# Autodesk Inventor assembly: PreliminaryDesignR1
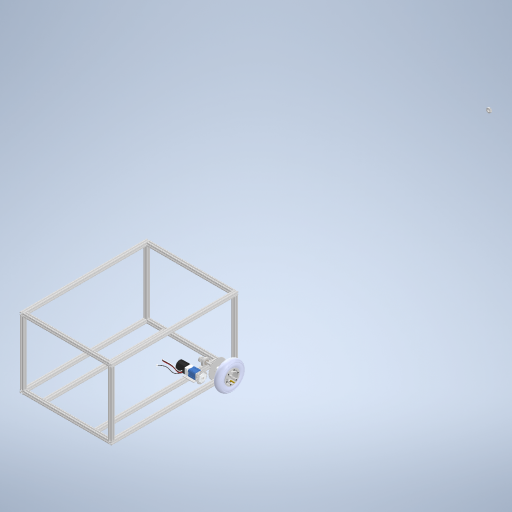
[picture p0: Inventor's stored thumbnail of the model, 512x512]
Saved by Autodesk Inventor 2023 (Build 270158000, 158)
## iProperties
Created: 2022-09-11
Part Number: PreliminaryDesignR1
Document SubType Name: Assembly
Designer: PC
Author: PC
## Documents named in this file (16)
- C:\Users\PC\Documents\PersonalCAD\ARCIGVC\IGVC-Robot\PreliminaryDesignR1.iam
- C:\Users\PC\Documents\PersonalCAD\ARCIGVC\IGVC-Robot\2ft80-20.ipt
- C:\Users\PC\Documents\PersonalCAD\ARCIGVC\IGVC-Robot\3ft80-20.ipt
- C:\Users\PC\Documents\PersonalCAD\ARCIGVC\IGVC-Robot\18in80-20.ipt
- C:\Users\PC\Documents\PersonalCAD\ARCIGVC\IGVC-Robot\34in80-20.ipt
- C:\Users\PC\Documents\PersonalCAD\ARCIGVC\IGVC-Robot\8inPneumatic.ipt
- C:\Users\PC\Documents\PersonalCAD\ARCIGVC\IGVC-Robot\2 Stage HD - CIM Sport.ipt
- C:\Users\PC\Documents\PersonalCAD\ARCIGVC\IGVC-Robot\am-4258 NEO Brushless Motor.ipt
- C:\Users\PC\Documents\PersonalCAD\ARCIGVC\IGVC-Robot\MotorMount.ipt
- C:\Users\PC\Documents\PersonalCAD\ARCIGVC\IGVC-Robot\24tSprocket35Series.ipt
- C:\Users\PC\Documents\PersonalCAD\ARCIGVC\IGVC-Robot\42tSprocket35Series.ipt
- C:\Users\PC\Documents\PersonalCAD\ARCIGVC\IGVC-Robot\Hex Hub .5In.ipt
- C:\Users\PC\Documents\PersonalCAD\ARCIGVC\IGVC-Robot\Bearing Housing.ipt
- C:\Users\PC\Documents\PersonalCAD\ARCIGVC\IGVC-Robot\HalfInHex Bearing.ipt
- C:\Users\PC\Documents\PersonalCAD\ARCIGVC\IGVC-Robot\9in-0.5inHexAxel.ipt
- C:\Users\PC\Documents\PersonalCAD\ARCIGVC\IGVC-Robot\am-1526 500Hex HD Collar Clamp.ipt
## Components (31 placed, 15 different names)
1. 2ft80-20:1 — Mate:1, Flush:1, Flush:2, Flush:4, Mate:4, Flush:7
2. 3ft80-20:1 — Mate:1, Flush:1, Flush:2, Mate:3, Flush:5, Flush:6, Mate:8, Flush:14, Flush:15, Mate:9, Flush:16, Flush:17
3. 2ft80-20:2 — Mate:3, Flush:5, Flush:6, Mate:13, Flush:24, Mate:14, Flush:25
4. 3ft80-20:2 — Flush:4, Mate:4, Flush:7, Mate:10, Flush:18, Flush:19, Mate:11, Flush:20, Flush:21, Mate:29, Flush:29, Mate:43, Mate:44, Mate:45
5. 2ft80-20:3
6. 3ft80-20:3
7. 2ft80-20:4
8. 3ft80-20:4 — Mate:12, Flush:22, Flush:23
9. 18in80-20:1 — Mate:8, Flush:14, Flush:15
10. 18in80-20:2 — Mate:9, Flush:16, Flush:17
11. 18in80-20:3 — Mate:11, Flush:20, Flush:21, Mate:12, Flush:22, Flush:23
12. 18in80-20:4 — Mate:10, Flush:18, Flush:19
13. 34in80-20:1 — Mate:13, Flush:24, Mate:21, Flush:26, Mate:30, Flush:28
14. 34in80-20:2 — Mate:14, Flush:25
15. 8inPneumatic:1 — Mate:41, Mate:43, Mate:45, Flush:31, Mate:48
16. 2 Stage HD - CIM Sport:1 — Mate:15, Mate:16, Mate:17, Mate:18, Mate:19, Mate:20, Mate:25, Flush:27, Mate:44
17. am-4258 NEO Brushless Motor:1 — Mate:15, Mate:16, Mate:17
18. MotorMount:1 — Mate:18, Mate:19, Mate:20, Mate:21, Flush:26, Mate:52
19. 24tSprocket35Series:1 — Mate:22, Mate:23, Mate:24, Flush:30
20. 42tSprocket35Series:1 — Mate:26, Mate:27, Mate:28, Flush:30
21. Hex Hub .5In:1 — Mate:26, Mate:27, Mate:28, Mate:42, Mate:46, Mate:47
22. Hex Hub .5In:2 — Mate:22, Mate:23, Mate:24, Mate:25, Flush:27
23. Bearing Housing:1 — Mate:29, Flush:29, Mate:31, Mate:32, Mate:33, Mate:35, Mate:36, Mate:41, Mate:42
24. Bearing Housing:2 — Mate:30, Flush:28, Mate:31, Mate:37, Mate:38, Mate:39, Mate:40, Mate:52
25. HalfInHex Bearing:1 — Mate:32, Mate:33
26. HalfInHex Bearing:2 — Mate:35, Mate:36
27. HalfInHex Bearing:3 — Mate:37, Mate:40
28. HalfInHex Bearing:4 — Mate:38, Mate:39
29. 9in-0.5inHexAxel:1 — Mate:46, Mate:47, Flush:31, Mate:48, Mate:50, Mate:51
30. am-1526 500Hex HD Collar Clamp:1
31. am-1526 500Hex HD Collar Clamp:2 — Mate:50, Mate:51
## Relationships (79: Mate 49, Flush 30)
- Mate:1: 2ft80-20:1 ↔ 3ft80-20:1
- Flush:1: 2ft80-20:1 ↔ 3ft80-20:1
- Flush:2: 2ft80-20:1 ↔ 3ft80-20:1
- Flush:4: 2ft80-20:1 ↔ 3ft80-20:2
- Mate:3: 3ft80-20:1 ↔ 2ft80-20:2
- Flush:5: 3ft80-20:1 ↔ 2ft80-20:2
- Flush:6: 3ft80-20:1 ↔ 2ft80-20:2
- Mate:4: 2ft80-20:1 ↔ 3ft80-20:2
- Flush:7: 2ft80-20:1 ↔ 3ft80-20:2
- [Mate]: 2ft80-20:3 ↔ 3ft80-20:3
- [Flush]: 2ft80-20:3 ↔ 3ft80-20:3
- [Flush]: 2ft80-20:3 ↔ 3ft80-20:3
- [Flush]: 2ft80-20:3 ↔ 3ft80-20:4
- [Mate]: 3ft80-20:3 ↔ 2ft80-20:4
- [Flush]: 3ft80-20:3 ↔ 2ft80-20:4
- [Flush]: 3ft80-20:3 ↔ 2ft80-20:4
- [Mate]: 2ft80-20:3 ↔ 3ft80-20:4
- [Flush]: 2ft80-20:3 ↔ 3ft80-20:4
- Mate:8: 3ft80-20:1 ↔ 18in80-20:1
- Flush:14: 3ft80-20:1 ↔ 18in80-20:1
- Flush:15: 3ft80-20:1 ↔ 18in80-20:1
- Mate:9: 3ft80-20:1 ↔ 18in80-20:2
- Flush:16: 3ft80-20:1 ↔ 18in80-20:2
- Flush:17: 3ft80-20:1 ↔ 18in80-20:2
- Mate:10: 3ft80-20:2 ↔ 18in80-20:4
- Flush:18: 3ft80-20:2 ↔ 18in80-20:4
- Flush:19: 3ft80-20:2 ↔ 18in80-20:4
- Mate:11: 3ft80-20:2 ↔ 18in80-20:3
- Flush:20: 3ft80-20:2 ↔ 18in80-20:3
- Flush:21: 3ft80-20:2 ↔ 18in80-20:3
- Mate:12: 3ft80-20:4 ↔ 18in80-20:3
- Flush:22: 3ft80-20:4 ↔ 18in80-20:3
- Flush:23: 3ft80-20:4 ↔ 18in80-20:3
- Mate:13: 2ft80-20:2 ↔ 34in80-20:1
- Flush:24: 2ft80-20:2 ↔ 34in80-20:1
- Mate:14: 2ft80-20:2 ↔ 34in80-20:2
- Flush:25: 2ft80-20:2 ↔ 34in80-20:2
- Mate:15: 2 Stage HD - CIM Sport:1 ↔ am-4258 NEO Brushless Motor:1
- Mate:16: 2 Stage HD - CIM Sport:1 ↔ am-4258 NEO Brushless Motor:1
- Mate:17: 2 Stage HD - CIM Sport:1 ↔ am-4258 NEO Brushless Motor:1
- Mate:18: 2 Stage HD - CIM Sport:1 ↔ MotorMount:1
- Mate:19: 2 Stage HD - CIM Sport:1 ↔ MotorMount:1
- Mate:20: 2 Stage HD - CIM Sport:1 ↔ MotorMount:1
- Mate:21: 34in80-20:1 ↔ MotorMount:1
- Flush:26: 34in80-20:1 ↔ MotorMount:1
- Mate:22: 24tSprocket35Series:1 ↔ Hex Hub .5In:2
- Mate:23: 24tSprocket35Series:1 ↔ Hex Hub .5In:2
- Mate:24: 24tSprocket35Series:1 ↔ Hex Hub .5In:2
- Mate:25: 2 Stage HD - CIM Sport:1 ↔ Hex Hub .5In:2
- Flush:27: 2 Stage HD - CIM Sport:1 ↔ Hex Hub .5In:2
- Mate:26: 42tSprocket35Series:1 ↔ Hex Hub .5In:1
- Mate:27: 42tSprocket35Series:1 ↔ Hex Hub .5In:1
- Mate:28: 42tSprocket35Series:1 ↔ Hex Hub .5In:1
- Mate:29: 3ft80-20:2 ↔ Bearing Housing:1
- Mate:30: 34in80-20:1 ↔ Bearing Housing:2
- Flush:28 (4.7625 mm): 34in80-20:1 ↔ Bearing Housing:2
- Flush:29 (4.7625 mm): 3ft80-20:2 ↔ Bearing Housing:1
- Mate:31: Bearing Housing:1 ↔ Bearing Housing:2
- Mate:32: Bearing Housing:1 ↔ HalfInHex Bearing:1
- Mate:33: Bearing Housing:1 ↔ HalfInHex Bearing:1
- Mate:35: Bearing Housing:1 ↔ HalfInHex Bearing:2
- Mate:36: Bearing Housing:1 ↔ HalfInHex Bearing:2
- Mate:37: Bearing Housing:2 ↔ HalfInHex Bearing:3
- Mate:38: Bearing Housing:2 ↔ HalfInHex Bearing:4
- Mate:39: Bearing Housing:2 ↔ HalfInHex Bearing:4
- Mate:40: Bearing Housing:2 ↔ HalfInHex Bearing:3
- Mate:41: 8inPneumatic:1 ↔ Bearing Housing:1
- Mate:42: Hex Hub .5In:1 ↔ Bearing Housing:1
- Flush:30: 24tSprocket35Series:1 ↔ 42tSprocket35Series:1
- Mate:43 (12.7 mm): 3ft80-20:2 ↔ 8inPneumatic:1
- Mate:44 (12.7 mm): 3ft80-20:2 ↔ 2 Stage HD - CIM Sport:1
- Mate:45 (-101.6 mm): 3ft80-20:2 ↔ 8inPneumatic:1
- Mate:46: Hex Hub .5In:1 ↔ 9in-0.5inHexAxel:1
- Mate:47: Hex Hub .5In:1 ↔ 9in-0.5inHexAxel:1
- Flush:31: 8inPneumatic:1 ↔ 9in-0.5inHexAxel:1
- Mate:48: 8inPneumatic:1 ↔ 9in-0.5inHexAxel:1
- Mate:50: 9in-0.5inHexAxel:1 ↔ am-1526 500Hex HD Collar Clamp:2
- Mate:51: 9in-0.5inHexAxel:1 ↔ am-1526 500Hex HD Collar Clamp:2
- Mate:52 (25.4 mm): MotorMount:1 ↔ Bearing Housing:2
## Named parameters: d11_d5 = 0 mm, d12_d6 = 0 mm, d13_d7 = 0 mm, d14_d8 = 0 mm, d15_d9 = 0 mm, d16_d10 = 0 mm, d17_d0 = 0 mm, d18_d1 = 0 mm, d19_d2 = 0 mm
